# Autodesk Inventor assembly: Cuarto
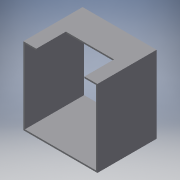
[picture p0: Inventor's stored thumbnail of the model, 180x180]
Saved by Autodesk Inventor 2016 (Build 200138000, 138)
## iProperties
Created: 2015-11-12
Part Number: Cuarto
Document SubType Name: Assembly
Designer: serge
Mass: 9.5758e+06 g
Surface Area: 3.83299e+06 cm^2
Volume: 9.5758e+06 cm^3
Density: 1 g/cm^3
Author: serge
## Documents named in this file (4)
- D:\Programas\xampp\htdocs\localUnal\storage\macros\cuarto\Modelado\Cuarto\Cuarto.iam
- D:\Programas\xampp\htdocs\localUnal\storage\macros\cuarto\Modelado\Cuarto\Pared ESTE Y OESTE.ipt
- D:\Programas\xampp\htdocs\localUnal\storage\macros\cuarto\Modelado\Cuarto\Pared Norte.ipt
- D:\Programas\xampp\htdocs\localUnal\storage\macros\cuarto\Modelado\Cuarto\Pared sur.ipt
## Components (4 placed, 3 different names)
1. Pared ESTE Y OESTE:1 — Mate:1, Flush:1, Flush:2
2. Pared Norte:1 — Mate:1, Flush:1, Flush:2, Mate:2, Flush:3, Flush:4
3. Pared sur:1 — Mate:3, Flush:5, Flush:6
4. Pared ESTE Y OESTE:2 — Mate:2, Flush:3, Flush:4, Mate:3, Flush:5, Flush:6
## Relationships (9: Flush 6, Mate 3)
- Mate:1: Pared ESTE Y OESTE:1 ↔ Pared Norte:1
- Flush:1: Pared ESTE Y OESTE:1 ↔ Pared Norte:1
- Flush:2: Pared ESTE Y OESTE:1 ↔ Pared Norte:1
- Mate:2: Pared Norte:1 ↔ Pared ESTE Y OESTE:2
- Flush:3: Pared Norte:1 ↔ Pared ESTE Y OESTE:2
- Flush:4: Pared Norte:1 ↔ Pared ESTE Y OESTE:2
- Mate:3: Pared sur:1 ↔ Pared ESTE Y OESTE:2
- Flush:5: Pared sur:1 ↔ Pared ESTE Y OESTE:2
- Flush:6: Pared sur:1 ↔ Pared ESTE Y OESTE:2
## Named parameters: primcon = 0 mm, secon = 0 mm, tercon = 0 mm, cuacon = 0 mm, quincon = 0 mm, sexcon = 0 mm, sepcon = 0 mm, octcon = 0 mm, novcon = 0 mm
